# Autodesk Inventor assembly: Kroller2
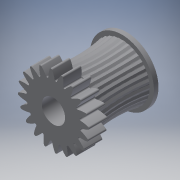
[picture p0: Inventor's stored thumbnail of the model, 180x180]
Saved by Autodesk Inventor 2016 (Build 200138000, 138)
## iProperties
Created: 2018-03-02
Part Number: Kroller2
Document SubType Name: Assembly
Designer: Simon
Author: Simon
## Documents named in this file (3)
- D:\Cad\Gymnasieprojekt\Kroller2.iam
- D:\Cad\Gymnasieprojekt\Kugg2.ipt
- D:\Cad\Gymnasieprojekt\Roller2_v3.ipt
## Components (2 placed, 2 different names)
1. Kugg2:1 — Insert:1
2. Roller2_v3:1 — Insert:1
## Relationships (1: Insert 1)
- Insert:1: Kugg2:1 ↔ Roller2_v3:1
